# Autodesk Inventor assembly: 6x1inTractionWheel.1111-2016
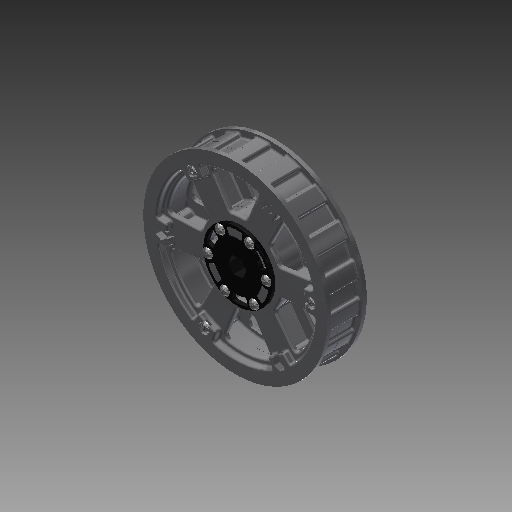
[picture p0: Inventor's stored thumbnail of the model, 512x512]
Saved by Autodesk Inventor 2017 (Build 210142000, 142)
## iProperties
Created: 2016-12-09
Part Number: 6x1inTractionWheel.1111-2016
Document SubType Name: Assembly
Designer: smiku
Author: smiku
## Documents named in this file (8)
- E:\GrabCAD\Power Hawks CAD\Resources\VEXpro Resources\Wheels\6 inch\6x1inTractionWheel-1111-2016.iam
- E:\GrabCAD\Power Hawks CAD\Resources\VEXpro Resources\Wheels\Wheel Parts\6InchWheelEnd-1111-2016.ipt
- E:\GrabCAD\Power Hawks CAD\Resources\VEXpro Resources\Fasteners\Standoffs\Standoff0.75in-1111-2016.ipt
- E:\GrabCAD\Power Hawks CAD\Resources\VEXpro Resources\Versa Motion\VersaHub(0.5inHex)-1111-2016.ipt
- E:\GrabCAD\Power Hawks CAD\Resources\VEXpro Resources\Versa Motion\VersaHub(0.5inHex,Plastic)-1111-2016.ipt
- E:\GrabCAD\Power Hawks CAD\Resources\VEXpro Resources\Fasteners\Screws\Screw8-32x1.25in-1111-2016.ipt
- E:\GrabCAD\Power Hawks CAD\Resources\VEXpro Resources\Fasteners\Screws\Screw8-32x0.5in-1111-2016.ipt
- E:\GrabCAD\Power Hawks CAD\Resources\VEXpro Resources\Fasteners\Nuts\Nut8-32Nylock-1111-2016.ipt
## Components (28 placed, 7 different names)
1. 6InchWheelEnd-1111-2016:1 — Rotational:1, Angle:1, Rotational:6, Rotational:7, Rotational:8, Rotational:9, Insert:16, Insert:17, Insert:18, Angle:2, Angle:3, Angle:4
2. 6InchWheelEnd-1111-2016:2 — Rotational:4, Rotational:5, Insert:1, Insert:2, Insert:3, Rotational:8, Rotational:9
3. VersaHub(0.5inHex)-1111-2016:1 — Rotational:4, Rotational:5, Insert:4, Insert:5, Insert:6, Insert:7, Insert:8, Insert:9
4. VersaHub(0.5inHex,Plastic)-1111-2016:1 — Rotational:6, Rotational:7, Insert:10, Insert:11, Insert:12, Insert:13, Insert:14, Insert:15
5. Screw8-32x1.25in-1111-2016:1 — Insert:1
6. Screw8-32x1.25in-1111-2016:2 — Insert:2
7. Screw8-32x1.25in-1111-2016:3 — Insert:3
8. Screw8-32x0.5in-1111-2016:1 — Insert:9
9. Screw8-32x0.5in-1111-2016:2 — Insert:8
10. Screw8-32x0.5in-1111-2016:3 — Insert:7
11. Screw8-32x0.5in-1111-2016:4 — Insert:6
12. Screw8-32x0.5in-1111-2016:5 — Insert:5
13. Screw8-32x0.5in-1111-2016:6 — Insert:4
14. Screw8-32x0.5in-1111-2016:7 — Insert:10
15. Screw8-32x0.5in-1111-2016:8 — Insert:11
16. Screw8-32x0.5in-1111-2016:9 — Insert:12
17. Screw8-32x0.5in-1111-2016:10 — Insert:13
18. Screw8-32x0.5in-1111-2016:11 — Insert:14
19. Screw8-32x0.5in-1111-2016:12 — Insert:15
20. Nut8-32Nylock-1111-2016:1 — Insert:17, Angle:3
21. Nut8-32Nylock-1111-2016:2 — Insert:16, Angle:4
22. Nut8-32Nylock-1111-2016:3 — Insert:18, Angle:2
23. Standoff0.75in-1111-2016:1 — Rotational:1, Angle:1
24. Standoff0.75in-1111-2016:2
25. Standoff0.75in-1111-2016:3
26. Standoff0.75in-1111-2016:4
27. Standoff0.75in-1111-2016:5
28. Standoff0.75in-1111-2016:6
## Component patterns: (6 elements, first: Standoff0.75in-1111-2016:1)
## Relationships (29: Insert 18, RevoluteJoint 7, Angle 4)
- Rotational:1 [RevoluteJoint]: 6InchWheelEnd-1111-2016:1 ↔ Standoff0.75in-1111-2016:1
- Angle:1 (0 deg): 6InchWheelEnd-1111-2016:1 ↔ Standoff0.75in-1111-2016:1
- Rotational:4 [RevoluteJoint]: 6InchWheelEnd-1111-2016:2 ↔ VersaHub(0.5inHex)-1111-2016:1
- Rotational:5 [RevoluteJoint]: 6InchWheelEnd-1111-2016:2 ↔ VersaHub(0.5inHex)-1111-2016:1
- Rotational:6 [RevoluteJoint]: 6InchWheelEnd-1111-2016:1 ↔ VersaHub(0.5inHex,Plastic)-1111-2016:1
- Rotational:7 [RevoluteJoint]: 6InchWheelEnd-1111-2016:1 ↔ VersaHub(0.5inHex,Plastic)-1111-2016:1
- Insert:1: 6InchWheelEnd-1111-2016:2 ↔ Screw8-32x1.25in-1111-2016:1
- Insert:2: 6InchWheelEnd-1111-2016:2 ↔ Screw8-32x1.25in-1111-2016:2
- Insert:3: 6InchWheelEnd-1111-2016:2 ↔ Screw8-32x1.25in-1111-2016:3
- Insert:4: VersaHub(0.5inHex)-1111-2016:1 ↔ Screw8-32x0.5in-1111-2016:6
- Insert:5: VersaHub(0.5inHex)-1111-2016:1 ↔ Screw8-32x0.5in-1111-2016:5
- Insert:6: VersaHub(0.5inHex)-1111-2016:1 ↔ Screw8-32x0.5in-1111-2016:4
- Insert:7: VersaHub(0.5inHex)-1111-2016:1 ↔ Screw8-32x0.5in-1111-2016:3
- Insert:8: VersaHub(0.5inHex)-1111-2016:1 ↔ Screw8-32x0.5in-1111-2016:2
- Insert:9: VersaHub(0.5inHex)-1111-2016:1 ↔ Screw8-32x0.5in-1111-2016:1
- Insert:10: VersaHub(0.5inHex,Plastic)-1111-2016:1 ↔ Screw8-32x0.5in-1111-2016:7
- Insert:11: VersaHub(0.5inHex,Plastic)-1111-2016:1 ↔ Screw8-32x0.5in-1111-2016:8
- Insert:12: VersaHub(0.5inHex,Plastic)-1111-2016:1 ↔ Screw8-32x0.5in-1111-2016:9
- Insert:13: VersaHub(0.5inHex,Plastic)-1111-2016:1 ↔ Screw8-32x0.5in-1111-2016:10
- Insert:14: VersaHub(0.5inHex,Plastic)-1111-2016:1 ↔ Screw8-32x0.5in-1111-2016:11
- Insert:15: VersaHub(0.5inHex,Plastic)-1111-2016:1 ↔ Screw8-32x0.5in-1111-2016:12
- Rotational:8 [RevoluteJoint]: 6InchWheelEnd-1111-2016:1 ↔ 6InchWheelEnd-1111-2016:2
- Rotational:9 [RevoluteJoint]: 6InchWheelEnd-1111-2016:1 ↔ 6InchWheelEnd-1111-2016:2
- Insert:16: 6InchWheelEnd-1111-2016:1 ↔ Nut8-32Nylock-1111-2016:2
- Insert:17: 6InchWheelEnd-1111-2016:1 ↔ Nut8-32Nylock-1111-2016:1
- Insert:18: 6InchWheelEnd-1111-2016:1 ↔ Nut8-32Nylock-1111-2016:3
- Angle:2 (0 deg): 6InchWheelEnd-1111-2016:1 ↔ Nut8-32Nylock-1111-2016:3
- Angle:3 (0 deg): 6InchWheelEnd-1111-2016:1 ↔ Nut8-32Nylock-1111-2016:1
- Angle:4 (0 deg): 6InchWheelEnd-1111-2016:1 ↔ Nut8-32Nylock-1111-2016:2
